# Autodesk Inventor assembly: 00_X02598_LEGOmini_CityGuy
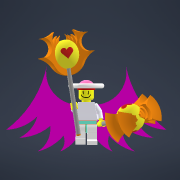
[picture p0: Inventor's stored thumbnail of the model, 180x180]
Saved by Autodesk Inventor 2022 (Build 260153000, 153)
## iProperties
Created: 2022-02-05
Part Number: 00_X02598_LEGOmini_CityGuy
Document SubType Name: Assembly
Designer: Jason
Author: Jason
## Documents named in this file (6)
- D:\D-disk\pomelo\大一\下學期\機械設計製圖\110033226_LEGOmini\110033226_LEGOmini_小人2\00_X02598_LEGOmini_CityGuy.iam
- D:\D-disk\pomelo\大一\下學期\機械設計製圖\110033226_LEGOmini\110033226_LEGOmini_小人2\X02598_LEGOmini_LowerBody.iam
- D:\D-disk\pomelo\大一\下學期\機械設計製圖\110033226_LEGOmini\110033226_LEGOmini_小人2\X02598_LEGOmini_UpperBody.iam
- D:\D-disk\pomelo\大一\下學期\機械設計製圖\110033226_LEGOmini\110033226_LEGOmini_小人2\X02598_LEGOmini_Head_Y.ipt
- D:\D-disk\pomelo\大一\下學期\機械設計製圖\110033226_LEGOmini\110033226_LEGOmini_小人2\X02598_LEGOmini_Hat_R.ipt
- D:\D-disk\pomelo\大一\下學期\機械設計製圖\110033226_LEGOmini\110033226_LEGOmini_小人2\110033226_LEGOmini_天使權杖.ipt
## Components (6 placed, 5 different names)
1. X02598_LEGOmini_LowerBody:1 [sub-assembly] — 貼合:1, 齊平:1, 齊平:2
2. X02598_LEGOmini_UpperBody:1 [sub-assembly] — 貼合:1, 齊平:1, 齊平:2, 插入:1, 貼合:2, 貼合:3
3. X02598_LEGOmini_Head_Y:1 — 插入:1, 插入:2
4. X02598_LEGOmini_Hat_R:1 — 插入:2
5. 110033226_LEGOmini_天使權杖:1 — 貼合:2
6. 110033226_LEGOmini_天使權杖:2 — 貼合:3
## Relationships (7: Mate 3, Flush 2, Insert 2)
- 貼合:1 [Mate]: X02598_LEGOmini_LowerBody:1 ↔ X02598_LEGOmini_UpperBody:1
- 齊平:1 [Flush]: X02598_LEGOmini_LowerBody:1 ↔ X02598_LEGOmini_UpperBody:1
- 齊平:2 [Flush]: X02598_LEGOmini_LowerBody:1 ↔ X02598_LEGOmini_UpperBody:1
- 插入:1 [Insert]: X02598_LEGOmini_UpperBody:1 ↔ X02598_LEGOmini_Head_Y:1
- 插入:2 [Insert]: X02598_LEGOmini_Head_Y:1 ↔ X02598_LEGOmini_Hat_R:1
- 貼合:2 [Mate]: X02598_LEGOmini_UpperBody:1 ↔ 110033226_LEGOmini_天使權杖:1
- 貼合:3 [Mate]: X02598_LEGOmini_UpperBody:1 ↔ 110033226_LEGOmini_天使權杖:2
